# Autodesk Inventor assembly: ABD_Version_0.1_leftleg
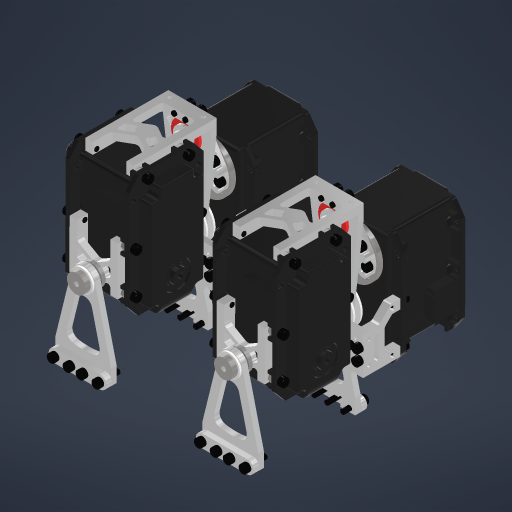
[picture p0: Inventor's stored thumbnail of the model, 512x512]
Saved by Autodesk Inventor 2024.3 (Build 283343000, 343)
## iProperties
Created: 2024-01-23
Part Number: ABD_Version_0.1_leftleg
Document SubType Name: Assembly
Designer: ASUS
Mass: 357.136 g
Surface Area: 604.848 cm^2
Volume: 181.423 cm^3
Density: 1.96853 g/cm^3
Author: ASUS
## Documents named in this file (27)
- C:\Users\ASUS\Desktop\Anti_Backlash_Structure_OP\v2_Frame\ABD_V2_Left_OP.iam
- C:\Users\ASUS\Desktop\Anti_Backlash_Structure_OP\v2_Frame\Roll_Fixation_Set.iam
- C:\Users\ASUS\Desktop\Anti_Backlash_Structure_OP\v2_Frame\ABD_MX_64_Roll_Fixation_Set.iam
- C:\Users\ASUS\Desktop\Anti_Backlash_Structure_OP\v2_Frame\ABD_MX_64_Slider_Fixation_Set_Right2Horn.iam
- C:\Users\ASUS\Desktop\Anti_Backlash_Structure_OP\v2_Frame\Roll_Fixation_Frame.ipt
- C:\Users\ASUS\Desktop\Anti_Backlash_Structure_OP\v2_Frame\Roll_Fixation_Frame_Back.ipt
- C:\Users\ASUS\Desktop\Anti_Backlash_Structure_OP\v2_Frame\hip joint fix washer.ipt
- C:\Users\ASUS\Desktop\Anti_Backlash_Structure_OP\MISUMI\hip_joint_fix_washer_10mm_Set.iam
- C:\Users\ASUS\Desktop\Anti_Backlash_Structure_OP\v2_Frame\Front_Frame_Fixer_v2.iam
- C:\Users\ASUS\Desktop\Anti_Backlash_Structure_OP\v2_Frame\Roll_Fixation_Frameto64.ipt
- C:\Users\ASUS\Desktop\Anti_Backlash_Structure_OP\MISUMI\CSH-ST-M2_5-6_203.ipt
- C:\Users\ASUS\Desktop\Anti_Backlash_Structure_OP\ROBOTIS(Inventor 2024 ver.)\DXL\MX-64T.ipt
- C:\Users\ASUS\Desktop\Anti_Backlash_Structure_OP\MISUMI\DBSY4-5-8.ipt
- C:\Users\ASUS\Desktop\Anti_Backlash_Structure_OP\MISUMI\C-WSSA12-4-2.ipt
- C:\Users\ASUS\Desktop\Anti_Backlash_Structure_OP\V2_Frame(2025)\MISUMI\TT-0822-10.ipt
- C:\Users\ASUS\Desktop\Anti_Backlash_Structure_OP\MISUMI\SLBNR4.ipt
- C:\Users\ASUS\Desktop\Anti_Backlash_Structure_OP\MISUMI\80F-0608.ipt
- C:\Users\ASUS\Desktop\Anti_Backlash_Structure_OP\MISUMI\E-GPWSSS8-4-1.ipt
- C:\Users\ASUS\Desktop\Anti_Backlash_Structure_OP\v2_Frame\M4-D6-10mm_Spacer.ipt
- C:\Users\ASUS\Desktop\Anti_Backlash_Structure_OP\V2_Frame(2025)\M4-18-low-head-bolt.ipt
- C:\Users\ASUS\Desktop\Anti_Backlash_Structure_OP\MISUMI\C-WSSA10-6-1.ipt
- C:\Users\ASUS\Desktop\Anti_Backlash_Structure_OP\v2_Frame\Crank_Slider_Fixer.iam
- C:\Users\ASUS\Desktop\2024_Robit_Hardware\ROBOCUP_2024_eindhoven\부품\ROBOTIS(Inventor 2023 ver.)\혼\64-106Horn.ipt
- C:\Users\ASUS\Desktop\Anti_Backlash_Structure_OP\v2_Frame\Slider_crank_horn_v2.ipt
- C:\Users\ASUS\Desktop\Anti_Backlash_Structure_OP\MISUMI\CSH-STN-M3-10_203.ipt
- C:\Users\ASUS\Desktop\Anti_Backlash_Structure_OP\MISUMI\4mm_ABD_set.iam
- C:\Users\ASUS\Desktop\Anti_Backlash_Structure_OP\MISUMI\TT-0409-05.ipt
## Components (47 placed, 26 different names)
1. Roll_Fixation_Set:1 [sub-assembly] — 삽입:5, 삽입:6, 각도:1, 플러쉬:7, 플러쉬:8, 메이트:43, 메이트:56
2. ABD_MX_64_Roll_Fixation_Set:1 [sub-assembly] — 메이트:2, 메이트:3, 삽입:5, 각도:1
3. ABD_MX_64_Slider_Fixation_Set_Right2Horn:1 [sub-assembly] — 메이트:2, 메이트:3, 삽입:6, 메이트:52, 메이트:53
4. SLBNR4:2 — 삽입:83, 각도:4
5. Roll_Fixation_Frame:2
6. Roll_Fixation_Frame_Back:2 — 메이트:45
7. hip joint fix washer:3
8. hip joint fix washer:4
9. hip_joint_fix_washer_10mm_Set:3 [sub-assembly]
10. hip_joint_fix_washer_10mm_Set:4 [sub-assembly]
11. Front_Frame_Fixer_v2:2 [sub-assembly] — 삽입:85
12. Roll_Fixation_Frameto64:3
13. Roll_Fixation_Frameto64:4
14. CSH-ST-M2_5-6_203:9
15. CSH-ST-M2_5-6_203:10
16. CSH-ST-M2_5-6_203:11
17. CSH-ST-M2_5-6_203:12
18. CSH-ST-M2_5-6_203:13
19. CSH-ST-M2_5-6_203:14
20. CSH-ST-M2_5-6_203:15
21. CSH-ST-M2_5-6_203:16
22. MX-64T:2 — 플러쉬:7, 플러쉬:8, 메이트:43, 메이트:55
23. DBSY4-5-8:2
24. ABD_MX_64_Roll_Fixation_Set:3 [sub-assembly] — 삽입:82, 각도:4, 메이트:46, 삽입:85
25. ABD_MX_64_Slider_Fixation_Set_Right2Horn:4 [sub-assembly] — 메이트:45, 메이트:46, 삽입:84, 메이트:51, 메이트:54
26. C-WSSA12-4-2:3 — 삽입:76, 삽입:82, 삽입:83, 삽입:87
27. TT-0822-10:3 — 삽입:77, 삽입:78, 삽입:84
28. 80F-0608:1 — 삽입:76, 삽입:77
29. TT-0822-10:4 — 삽입:78
30. M4-D6-10mm_Spacer:1 — 삽입:87, 삽입:89
31. M4-18-low-head-bolt:1 — 삽입:88
32. E-GPWSSS12-4-1:1 — 삽입:88, 삽입:89, 삽입:90
33. C-WSSA10-6-1:1 — 삽입:90
34. Crank_Slider_Fixer:5 [sub-assembly] — 삽입:100, 메이트:51, 메이트:54
35. 64-106Horn:1 — 삽입:96, 메이트:47, 삽입:98
36. CSH-STN-M3-10_203:1 — 메이트:55
37. 4mm_ABD_set:1 [sub-assembly] — 삽입:96, 메이트:47, 메이트:48
38. TT-0409-05:1 — 삽입:97, 삽입:99
39. M4-18-low-head-bolt:2 — 삽입:97
40. Slider_crank_horn_v2:1 — 삽입:98, 메이트:48, 삽입:99, 삽입:100
41. Crank_Slider_Fixer:6 [sub-assembly] — 메이트:52, 메이트:53
42. 64-106Horn:2
43. CSH-STN-M3-10_203:2 — 메이트:56
44. 4mm_ABD_set:2 [sub-assembly]
45. TT-0409-05:2
46. M4-18-low-head-bolt:3
47. Slider_crank_horn_v2:2
## Relationships (77: Insert 44, Mate 28, Angle 3, Flush 2)
- 메이트:2 [Mate] (0.05 mm): ABD_MX_64_Roll_Fixation_Set:1 ↔ ABD_MX_64_Slider_Fixation_Set_Right2Horn:1
- 메이트:3 [Mate]: ABD_MX_64_Roll_Fixation_Set:1 ↔ ABD_MX_64_Slider_Fixation_Set_Right2Horn:1
- 삽입:5 [Insert]: Roll_Fixation_Set:1 ↔ ABD_MX_64_Roll_Fixation_Set:1
- 삽입:6 [Insert]: Roll_Fixation_Set:1 ↔ ABD_MX_64_Slider_Fixation_Set_Right2Horn:1
- 각도:1 [Angle] (0 deg): Roll_Fixation_Set:1 ↔ ABD_MX_64_Roll_Fixation_Set:1
- [Mate]: Roll_Fixation_Frame:2 ↔ Roll_Fixation_Frame_Back:2
- [Insert]: Roll_Fixation_Frame:2 ↔ hip joint fix washer:3
- [Insert]: Roll_Fixation_Frame:2 ↔ hip joint fix washer:3
- [Insert]: Roll_Fixation_Frame_Back:2 ↔ hip joint fix washer:4
- [Mate]: Roll_Fixation_Frame_Back:2 ↔ hip joint fix washer:4
- [Mate]: Roll_Fixation_Frame_Back:2 ↔ hip joint fix washer:3
- [Mate]: Roll_Fixation_Frame_Back:2 ↔ hip joint fix washer:3
- [Mate]: Roll_Fixation_Frame:2 ↔ hip joint fix washer:3
- [Insert]: hip joint fix washer:3 ↔ hip_joint_fix_washer_10mm_Set:3
- [Mate]: hip joint fix washer:3 ↔ hip_joint_fix_washer_10mm_Set:3
- [Insert]: hip joint fix washer:4 ↔ hip_joint_fix_washer_10mm_Set:4
- [Mate]: hip joint fix washer:4 ↔ hip_joint_fix_washer_10mm_Set:4
- [Mate] (49 mm): Roll_Fixation_Frame:2 ↔ Roll_Fixation_Frame_Back:2
- [Mate]: hip_joint_fix_washer_10mm_Set:3 ↔ hip_joint_fix_washer_10mm_Set:4
- [Mate]: hip_joint_fix_washer_10mm_Set:3 ↔ hip_joint_fix_washer_10mm_Set:4
- [Insert]: Roll_Fixation_Frame_Back:2 ↔ Roll_Fixation_Frameto64:4
- [Insert]: Roll_Fixation_Frame_Back:2 ↔ Roll_Fixation_Frameto64:3
- [Mate]: Roll_Fixation_Frame_Back:2 ↔ Roll_Fixation_Frameto64:4
- [Mate]: Roll_Fixation_Frame_Back:2 ↔ Roll_Fixation_Frameto64:3
- [Insert]: Roll_Fixation_Frame_Back:2 ↔ CSH-ST-M2_5-6_203:10
- [Insert]: Roll_Fixation_Frame_Back:2 ↔ CSH-ST-M2_5-6_203:9
- [Insert]: Roll_Fixation_Frame_Back:2 ↔ CSH-ST-M2_5-6_203:11
- [Insert]: Roll_Fixation_Frame_Back:2 ↔ CSH-ST-M2_5-6_203:12
- [Insert] (2.5 mm): Roll_Fixation_Frameto64:4 ↔ CSH-ST-M2_5-6_203:15
- [Insert] (2.5 mm): Roll_Fixation_Frameto64:3 ↔ CSH-ST-M2_5-6_203:14
- [Insert] (2.5 mm): Roll_Fixation_Frameto64:3 ↔ CSH-ST-M2_5-6_203:13
- [Insert] (2.5 mm): Roll_Fixation_Frameto64:4 ↔ CSH-ST-M2_5-6_203:16
- [Insert]: Roll_Fixation_Frameto64:3 ↔ MX-64T:2
- [Insert]: Roll_Fixation_Frameto64:3 ↔ MX-64T:2
- [Insert]: Front_Frame_Fixer_v2:2 ↔ DBSY4-5-8:2
- [Insert]: Roll_Fixation_Frame:2 ↔ Front_Frame_Fixer_v2:2
- [Mate]: ABD_MX_64_Roll_Fixation_Set:3 ↔ ABD_MX_64_Slider_Fixation_Set_Right2Horn:4
- [Angle] (0 deg): MX-64T:2 ↔ ABD_MX_64_Roll_Fixation_Set:3
- 플러쉬:7 [Flush]: Roll_Fixation_Set:1 ↔ MX-64T:2
- 플러쉬:8 [Flush]: Roll_Fixation_Set:1 ↔ MX-64T:2
- 메이트:43 [Mate] (50 mm): Roll_Fixation_Set:1 ↔ MX-64T:2
- 삽입:76 [Insert]: C-WSSA12-4-2:3 ↔ 80F-0608:1
- 삽입:77 [Insert] (3 mm): TT-0822-10:3 ↔ 80F-0608:1
- 삽입:78 [Insert] (3 mm): TT-0822-10:3 ↔ TT-0822-10:4
- 메이트:45 [Mate]: Roll_Fixation_Frame_Back:2 ↔ ABD_MX_64_Slider_Fixation_Set_Right2Horn:4
- 삽입:82 [Insert]: ABD_MX_64_Roll_Fixation_Set:3 ↔ C-WSSA12-4-2:3
- 삽입:83 [Insert] (1 mm): SLBNR4:2 ↔ C-WSSA12-4-2:3
- 각도:4 [Angle] (0 deg): SLBNR4:2 ↔ ABD_MX_64_Roll_Fixation_Set:3
- 메이트:46 [Mate]: ABD_MX_64_Roll_Fixation_Set:3 ↔ ABD_MX_64_Slider_Fixation_Set_Right2Horn:4
- 삽입:84 [Insert]: ABD_MX_64_Slider_Fixation_Set_Right2Horn:4 ↔ TT-0822-10:3
- 삽입:85 [Insert]: Front_Frame_Fixer_v2:2 ↔ ABD_MX_64_Roll_Fixation_Set:3
- 삽입:87 [Insert]: C-WSSA12-4-2:3 ↔ M4-D6-10mm_Spacer:1
- 삽입:88 [Insert]: M4-18-low-head-bolt:1 ↔ E-GPWSSS12-4-1:1
- 삽입:89 [Insert]: M4-D6-10mm_Spacer:1 ↔ E-GPWSSS12-4-1:1
- 삽입:90 [Insert]: E-GPWSSS12-4-1:1 ↔ C-WSSA10-6-1:1
- [Insert]: 64-106Horn:1 ↔ CSH-STN-M3-10_203:1
- 삽입:96 [Insert] (2 mm): 64-106Horn:1 ↔ 4mm_ABD_set:1
- 메이트:47 [Mate]: 64-106Horn:1 ↔ 4mm_ABD_set:1
- 삽입:97 [Insert]: TT-0409-05:1 ↔ M4-18-low-head-bolt:2
- 삽입:98 [Insert]: 64-106Horn:1 ↔ Slider_crank_horn_v2:1
- 메이트:48 [Mate]: 4mm_ABD_set:1 ↔ Slider_crank_horn_v2:1
- 삽입:99 [Insert]: TT-0409-05:1 ↔ Slider_crank_horn_v2:1
- 삽입:100 [Insert]: Crank_Slider_Fixer:5 ↔ Slider_crank_horn_v2:1
- [Insert]: 64-106Horn:2 ↔ CSH-STN-M3-10_203:2
- [Insert] (2 mm): 64-106Horn:2 ↔ 4mm_ABD_set:2
- [Mate]: 64-106Horn:2 ↔ 4mm_ABD_set:2
- [Insert]: TT-0409-05:2 ↔ M4-18-low-head-bolt:3
- [Insert]: 64-106Horn:2 ↔ Slider_crank_horn_v2:2
- [Mate]: 4mm_ABD_set:2 ↔ Slider_crank_horn_v2:2
- [Insert]: TT-0409-05:2 ↔ Slider_crank_horn_v2:2
- [Insert]: Crank_Slider_Fixer:6 ↔ Slider_crank_horn_v2:2
- 메이트:51 [Mate]: ABD_MX_64_Slider_Fixation_Set_Right2Horn:4 ↔ Crank_Slider_Fixer:5
- 메이트:52 [Mate]: ABD_MX_64_Slider_Fixation_Set_Right2Horn:1 ↔ Crank_Slider_Fixer:6
- 메이트:53 [Mate]: ABD_MX_64_Slider_Fixation_Set_Right2Horn:1 ↔ Crank_Slider_Fixer:6
- 메이트:54 [Mate]: ABD_MX_64_Slider_Fixation_Set_Right2Horn:4 ↔ Crank_Slider_Fixer:5
- 메이트:55 [Mate]: MX-64T:2 ↔ CSH-STN-M3-10_203:1
- 메이트:56 [Mate]: Roll_Fixation_Set:1 ↔ CSH-STN-M3-10_203:2
## Named parameters: d1064_d1048 = 0 mm, d1072_d1058 = 0 deg, d1075_d838 = 0 mm, d1076_d839 = 0 mm, d1077_d840 = 0 mm, d1078_d841 = 0 mm, d1079_d587 = 0 mm, d1080_d753 = 0 mm, d1081_d754 = 0 mm, d1082_d756 = 0 mm, d1083_d757 = 0 mm, d1084_d761 = 0 mm, d1085_d762 = 0 mm, d1086_d764 = 0 mm, d1087_d49 = 0 mm, d1088_d50 = 0 mm, d1089_d16 = 49 mm, d1090_d17 = 0 mm, d1091_d18 = 0 mm, d1092_d20 = 0 mm, d1093_d21 = 0 mm, d1094_d22 = 0 mm, d1095_d23 = 0 mm, d1096_d24 = 0 mm, d1097_d25 = 0 mm, d1098_d26 = 0 mm, d1099_d27 = 0 mm, d1100_d31 = 2.5 mm, d1101_d32 = 2.5 mm, d1102_d33 = 2.5 mm, d1103_d34 = 2.5 mm, d1104_d35 = 0 mm, d1105_d36 = 0 mm, d1148_d4 = 0 mm, d1149_d1141 = 2 mm, d1150_d1142 = 0 mm, d1151_d1143 = 0 mm, d1152_d1144 = 0 mm, d1153_d1145 = 0 mm, d1154_d1146 = 0 mm, d1155_d1147 = 0 mm
